# Autodesk Inventor assembly: robot_main_board
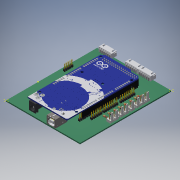
[picture p0: Inventor's stored thumbnail of the model, 180x180]
Saved by Autodesk Inventor 2019 (Build 230136000, 136)
## iProperties
Created: 2020-01-04
Part Number: robot_main_board
Material: Типовые
Document SubType Name: Assembly
Designer: Петров Иван
Author: Петров Иван
## Documents named in this file (7)
- E:\IVAN\Ivan_desktop\GitHub\Arm_manip\electronic\3d_visualization\robot_main_board\robot_main_board.iam
- E:\IVAN\Ivan_desktop\GitHub\Arm_manip\electronic\3d_visualization\robot_main_board\board.ipt
- E:\IVAN\Ivan_desktop\GitHub\Arm_manip\electronic\3d_visualization\lib\Connectors\PLS-1_(DS1021_CONNFLY).ipt
- E:\IVAN\Ivan_desktop\GitHub\Arm_manip\electronic\3d_visualization\lib\resistors\1,0 kOhm R Axial DIN0207 L6.3mm D2.5mm P7.62mm Horizontal.ipt
- E:\IVAN\Ivan_desktop\GitHub\Arm_manip\electronic\3d_visualization\lib\Connectors\JST - XH - Thru (R) - 6Pin - 2.54mm.ipt
- E:\IVAN\Ivan_desktop\GitHub\Arm_manip\electronic\3d_visualization\lib\Connectors\Molex 22-27-2021 v1.ipt
- E:\IVAN\Ivan_desktop\GitHub\Arm_manip\electronic\3d_visualization\lib\Arduino MEGA 2560 R3.ipt
## Components (151 placed, 6 different names)
1. board:1 — Совмещение:1, Совмещение:2, Угол:1, Совмещение:3, Совмещение:4, Совмещение:5, Совмещение:6, Совмещение:7, Совмещение:8, Угол:4, Угол:5, Угол:6, Совмещение:9, Совмещение:10, Угол:7, Совмещение:11, Совмещение:12, Угол:8, Совмещение:13, Угол:9, Совмещение:14, Совмещение:15, Угол:10, Совмещение:16, Совмещение:17, Угол:11, Совмещение:18, Совмещение:19, Совмещение:20, Совмещение:21, Угол:13, Совмещение:22, Совмещение:23, Угол:14, Совмещение:24, Совмещение:25, Совмещение:26, Угол:15, Совмещение:27, Угол:16, Совмещение:28, Совмещение:29, Совмещение:30, Касательность:1, Совмещение:31, Совмещение:32, Касательность:2, Совмещение:33, Совмещение:34, Касательность:3, Совмещение:35, Совмещение:36, Касательность:4, Совмещение:37, Совмещение:38, Касательность:5, Совмещение:39, Совмещение:40, Касательность:6, Совмещение:41, Совмещение:42, Касательность:7, Совмещение:43, Совмещение:44, Касательность:8, Совмещение:45, Совмещение:46, Совмещение:47, Совмещение:48, Совмещение:49, Совмещение:50, Совмещение:51, Совмещение:52, Совмещение:53, Совмещение:54, Совмещение:55, Угол:17, Совмещение:56, Угол:18, Совмещение:57, Совмещение:58, Совмещение:59, Совмещение:60, Совмещение:61, Совмещение:62, Совмещение:63, Угол:19, Угол:20, Угол:21, Угол:22, Угол:23, Угол:24, Совмещение:64, Совмещение:65, Совмещение:66, Совмещение:67, Совмещение:68, Совмещение:69
2. 1,0 kOhm R Axial DIN0207 L6.3mm D2.5mm P7.62mm Horizontal:1 — Совмещение:29, Совмещение:30, Касательность:1
3. 1,0 kOhm R Axial DIN0207 L6.3mm D2.5mm P7.62mm Horizontal:2 — Совмещение:31, Совмещение:32, Касательность:2
4. 1,0 kOhm R Axial DIN0207 L6.3mm D2.5mm P7.62mm Horizontal:3 — Совмещение:33, Совмещение:34, Касательность:3
5. 1,0 kOhm R Axial DIN0207 L6.3mm D2.5mm P7.62mm Horizontal:4 — Совмещение:35, Совмещение:36, Касательность:4
6. 1,0 kOhm R Axial DIN0207 L6.3mm D2.5mm P7.62mm Horizontal:5 — Совмещение:37, Совмещение:38, Касательность:5
7. 1,0 kOhm R Axial DIN0207 L6.3mm D2.5mm P7.62mm Horizontal:6 — Совмещение:39, Совмещение:40, Касательность:6
8. 1,0 kOhm R Axial DIN0207 L6.3mm D2.5mm P7.62mm Horizontal:7 — Совмещение:41, Совмещение:42, Касательность:7
9. 1,0 kOhm R Axial DIN0207 L6.3mm D2.5mm P7.62mm Horizontal:8 — Совмещение:43, Совмещение:44, Касательность:8
10. JST - XH - Thru (R) - 6Pin - 2.54mm:1 — Совмещение:51, Совмещение:52, Совмещение:53
11. JST - XH - Thru (R) - 6Pin - 2.54mm:2 — Совмещение:48, Совмещение:49, Совмещение:50
12. JST - XH - Thru (R) - 6Pin - 2.54mm:3 — Совмещение:45, Совмещение:46, Совмещение:47
13. Molex 22-27-2021 v1:1 — Совмещение:54, Совмещение:55, Угол:17
14. Molex 22-27-2021 v1:2 — Совмещение:56, Угол:18, Совмещение:57
15. Molex 22-27-2021 v1:3 — Совмещение:58, Угол:24, Совмещение:64
16. Molex 22-27-2021 v1:4 — Совмещение:59, Угол:23, Совмещение:65
17. Molex 22-27-2021 v1:5 — Совмещение:60, Угол:22, Совмещение:66
18. Molex 22-27-2021 v1:6 — Совмещение:61, Угол:21, Совмещение:67
19. Molex 22-27-2021 v1:7 — Совмещение:62, Угол:19, Совмещение:68
20. Molex 22-27-2021 v1:8 — Совмещение:63, Угол:20, Совмещение:69
21. Arduino MEGA 2560 R3:1 — Совмещение:70, Совмещение:72, Совмещение:73
22. PLS-1_(DS1021_CONNFLY):1 — Совмещение:1, Совмещение:2, Угол:1
23. PLS-1_(DS1021_CONNFLY):4
24. PLS-1_(DS1021_CONNFLY):5
25. PLS-1_(DS1021_CONNFLY):6
26. PLS-1_(DS1021_CONNFLY):7
27. PLS-1_(DS1021_CONNFLY):2 — Совмещение:3, Совмещение:4, Угол:5
28. PLS-1_(DS1021_CONNFLY):8
29. PLS-1_(DS1021_CONNFLY):9
30. PLS-1_(DS1021_CONNFLY):10
31. PLS-1_(DS1021_CONNFLY):11
32. PLS-1_(DS1021_CONNFLY):12
33. PLS-1_(DS1021_CONNFLY):13
34. PLS-1_(DS1021_CONNFLY):3 — Совмещение:5, Совмещение:6, Угол:6
35. PLS-1_(DS1021_CONNFLY):14
36. PLS-1_(DS1021_CONNFLY):15
37. PLS-1_(DS1021_CONNFLY):16
38. PLS-1_(DS1021_CONNFLY):17
39. PLS-1_(DS1021_CONNFLY):18 — Совмещение:7, Совмещение:8, Угол:4
40. PLS-1_(DS1021_CONNFLY):19
41. PLS-1_(DS1021_CONNFLY):20
42. PLS-1_(DS1021_CONNFLY):21
43. PLS-1_(DS1021_CONNFLY):22
44. PLS-1_(DS1021_CONNFLY):23 — Совмещение:9, Совмещение:10, Угол:7
45. PLS-1_(DS1021_CONNFLY):33
46. PLS-1_(DS1021_CONNFLY):34
47. PLS-1_(DS1021_CONNFLY):35
48. PLS-1_(DS1021_CONNFLY):36
49. PLS-1_(DS1021_CONNFLY):37
50. PLS-1_(DS1021_CONNFLY):38
51. PLS-1_(DS1021_CONNFLY):39
52. PLS-1_(DS1021_CONNFLY):24 — Совмещение:11, Совмещение:12, Угол:8
53. PLS-1_(DS1021_CONNFLY):40
54. PLS-1_(DS1021_CONNFLY):41
55. PLS-1_(DS1021_CONNFLY):42
56. PLS-1_(DS1021_CONNFLY):43
57. PLS-1_(DS1021_CONNFLY):44
58. PLS-1_(DS1021_CONNFLY):45
59. PLS-1_(DS1021_CONNFLY):46
60. PLS-1_(DS1021_CONNFLY):25 — Совмещение:13, Угол:9, Совмещение:14
61. PLS-1_(DS1021_CONNFLY):47
62. PLS-1_(DS1021_CONNFLY):48
63. PLS-1_(DS1021_CONNFLY):49
64. PLS-1_(DS1021_CONNFLY):50
65. PLS-1_(DS1021_CONNFLY):51
66. PLS-1_(DS1021_CONNFLY):52
67. PLS-1_(DS1021_CONNFLY):53
68. PLS-1_(DS1021_CONNFLY):26 — Совмещение:15, Угол:10, Совмещение:16
69. PLS-1_(DS1021_CONNFLY):54
70. PLS-1_(DS1021_CONNFLY):55
71. PLS-1_(DS1021_CONNFLY):56
72. PLS-1_(DS1021_CONNFLY):57
73. PLS-1_(DS1021_CONNFLY):58
74. PLS-1_(DS1021_CONNFLY):59
75. PLS-1_(DS1021_CONNFLY):60
76. PLS-1_(DS1021_CONNFLY):61
77. PLS-1_(DS1021_CONNFLY):62
78. PLS-1_(DS1021_CONNFLY):63
79. PLS-1_(DS1021_CONNFLY):64
80. PLS-1_(DS1021_CONNFLY):65
81. PLS-1_(DS1021_CONNFLY):66
82. PLS-1_(DS1021_CONNFLY):67
83. PLS-1_(DS1021_CONNFLY):68
84. PLS-1_(DS1021_CONNFLY):69
85. PLS-1_(DS1021_CONNFLY):70
86. PLS-1_(DS1021_CONNFLY):71
87. PLS-1_(DS1021_CONNFLY):72
88. PLS-1_(DS1021_CONNFLY):73
89. PLS-1_(DS1021_CONNFLY):74
90. PLS-1_(DS1021_CONNFLY):75
91. PLS-1_(DS1021_CONNFLY):76
92. PLS-1_(DS1021_CONNFLY):77
93. PLS-1_(DS1021_CONNFLY):78
94. PLS-1_(DS1021_CONNFLY):79
95. PLS-1_(DS1021_CONNFLY):80
96. PLS-1_(DS1021_CONNFLY):81
97. PLS-1_(DS1021_CONNFLY):82
98. PLS-1_(DS1021_CONNFLY):83
99. PLS-1_(DS1021_CONNFLY):84
100. PLS-1_(DS1021_CONNFLY):85
101. PLS-1_(DS1021_CONNFLY):86
102. PLS-1_(DS1021_CONNFLY):87
103. PLS-1_(DS1021_CONNFLY):88 — Совмещение:73
104. PLS-1_(DS1021_CONNFLY):27 — Совмещение:17, Угол:11, Совмещение:18, Угол:12, Совмещение:70
105. PLS-1_(DS1021_CONNFLY):28 — Совмещение:19, Угол:12, Совмещение:20
106. PLS-1_(DS1021_CONNFLY):30 — Совмещение:23, Угол:14, Совмещение:24
107. PLS-1_(DS1021_CONNFLY):29 — Совмещение:21, Угол:13, Совмещение:22
108. PLS-1_(DS1021_CONNFLY):89
109. PLS-1_(DS1021_CONNFLY):90
110. PLS-1_(DS1021_CONNFLY):103
111. PLS-1_(DS1021_CONNFLY):110
112. PLS-1_(DS1021_CONNFLY):91
113. PLS-1_(DS1021_CONNFLY):92
114. PLS-1_(DS1021_CONNFLY):104
115. PLS-1_(DS1021_CONNFLY):111
116. PLS-1_(DS1021_CONNFLY):93
117. PLS-1_(DS1021_CONNFLY):94
118. PLS-1_(DS1021_CONNFLY):105
119. PLS-1_(DS1021_CONNFLY):112
120. PLS-1_(DS1021_CONNFLY):95
121. PLS-1_(DS1021_CONNFLY):96
122. PLS-1_(DS1021_CONNFLY):106
123. PLS-1_(DS1021_CONNFLY):113
124. PLS-1_(DS1021_CONNFLY):97
125. PLS-1_(DS1021_CONNFLY):98
126. PLS-1_(DS1021_CONNFLY):107
127. PLS-1_(DS1021_CONNFLY):114
128. PLS-1_(DS1021_CONNFLY):99
129. PLS-1_(DS1021_CONNFLY):100
130. PLS-1_(DS1021_CONNFLY):108
131. PLS-1_(DS1021_CONNFLY):115
132. PLS-1_(DS1021_CONNFLY):101
133. PLS-1_(DS1021_CONNFLY):102
134. PLS-1_(DS1021_CONNFLY):109
135. PLS-1_(DS1021_CONNFLY):116
136. PLS-1_(DS1021_CONNFLY):31 — Совмещение:25, Совмещение:26, Угол:15
137. PLS-1_(DS1021_CONNFLY):117
138. PLS-1_(DS1021_CONNFLY):118
139. PLS-1_(DS1021_CONNFLY):119
140. PLS-1_(DS1021_CONNFLY):120
141. PLS-1_(DS1021_CONNFLY):121
142. PLS-1_(DS1021_CONNFLY):122
143. PLS-1_(DS1021_CONNFLY):123
144. PLS-1_(DS1021_CONNFLY):124
145. PLS-1_(DS1021_CONNFLY):125 — Совмещение:72
146. PLS-1_(DS1021_CONNFLY):32 — Совмещение:27, Угол:16, Совмещение:28
147. PLS-1_(DS1021_CONNFLY):126
148. PLS-1_(DS1021_CONNFLY):127
149. PLS-1_(DS1021_CONNFLY):128
150. PLS-1_(DS1021_CONNFLY):129
151. PLS-1_(DS1021_CONNFLY):130
## Component patterns: (5 elements, first: PLS-1_(DS1021_CONNFLY):1), (7 elements, first: PLS-1_(DS1021_CONNFLY):2), (5 elements, first: PLS-1_(DS1021_CONNFLY):3), (5 elements, first: PLS-1_(DS1021_CONNFLY):18), (8 elements, first: PLS-1_(DS1021_CONNFLY):23), (8 elements, first: PLS-1_(DS1021_CONNFLY):24), (8 elements, first: PLS-1_(DS1021_CONNFLY):25), (36 elements, first: PLS-1_(DS1021_CONNFLY):26), (8 elements, first: PLS-1_(DS1021_CONNFLY):27 + PLS-1_(DS1021_CONNFLY):28 + PLS-1_(DS1021_CONNFLY):30 + PLS-1_(DS1021_CONNFLY):29), (10 elements, first: PLS-1_(DS1021_CONNFLY):31), (6 elements, first: PLS-1_(DS1021_CONNFLY):32)
## Relationships (102: Mate 72, Angle 22, Tangent 8)
- Совмещение:1 [Mate]: board:1 ↔ PLS-1_(DS1021_CONNFLY):1
- Совмещение:2 [Mate]: board:1 ↔ PLS-1_(DS1021_CONNFLY):1
- Угол:1 [Angle] (90 deg): board:1 ↔ PLS-1_(DS1021_CONNFLY):1
- Совмещение:3 [Mate]: board:1 ↔ PLS-1_(DS1021_CONNFLY):2
- Совмещение:4 [Mate]: board:1 ↔ PLS-1_(DS1021_CONNFLY):2
- Совмещение:5 [Mate]: board:1 ↔ PLS-1_(DS1021_CONNFLY):3
- Совмещение:6 [Mate]: board:1 ↔ PLS-1_(DS1021_CONNFLY):3
- Совмещение:7 [Mate]: board:1 ↔ PLS-1_(DS1021_CONNFLY):18
- Совмещение:8 [Mate]: board:1 ↔ PLS-1_(DS1021_CONNFLY):18
- Угол:4 [Angle] (90 deg): board:1 ↔ PLS-1_(DS1021_CONNFLY):18
- Угол:5 [Angle] (90 deg): board:1 ↔ PLS-1_(DS1021_CONNFLY):2
- Угол:6 [Angle] (90 deg): board:1 ↔ PLS-1_(DS1021_CONNFLY):3
- Совмещение:9 [Mate]: board:1 ↔ PLS-1_(DS1021_CONNFLY):23
- Совмещение:10 [Mate]: board:1 ↔ PLS-1_(DS1021_CONNFLY):23
- Угол:7 [Angle] (0 deg): board:1 ↔ PLS-1_(DS1021_CONNFLY):23
- Совмещение:11 [Mate]: board:1 ↔ PLS-1_(DS1021_CONNFLY):24
- Совмещение:12 [Mate]: board:1 ↔ PLS-1_(DS1021_CONNFLY):24
- Угол:8 [Angle] (0 deg): board:1 ↔ PLS-1_(DS1021_CONNFLY):24
- Совмещение:13 [Mate]: board:1 ↔ PLS-1_(DS1021_CONNFLY):25
- Угол:9 [Angle] (0 deg): board:1 ↔ PLS-1_(DS1021_CONNFLY):25
- Совмещение:14 [Mate]: board:1 ↔ PLS-1_(DS1021_CONNFLY):25
- Совмещение:15 [Mate]: board:1 ↔ PLS-1_(DS1021_CONNFLY):26
- Угол:10 [Angle] (90 deg): board:1 ↔ PLS-1_(DS1021_CONNFLY):26
- Совмещение:16 [Mate]: board:1 ↔ PLS-1_(DS1021_CONNFLY):26
- Совмещение:17 [Mate]: board:1 ↔ PLS-1_(DS1021_CONNFLY):27
- Угол:11 [Angle] (0 deg): board:1 ↔ PLS-1_(DS1021_CONNFLY):27
- Совмещение:18 [Mate]: board:1 ↔ PLS-1_(DS1021_CONNFLY):27
- Совмещение:19 [Mate]: board:1 ↔ PLS-1_(DS1021_CONNFLY):28
- Угол:12 [Angle] (90 deg): PLS-1_(DS1021_CONNFLY):27 ↔ PLS-1_(DS1021_CONNFLY):28
- Совмещение:20 [Mate]: board:1 ↔ PLS-1_(DS1021_CONNFLY):28
- Совмещение:21 [Mate]: board:1 ↔ PLS-1_(DS1021_CONNFLY):29
- Угол:13 [Angle] (90 deg): board:1 ↔ PLS-1_(DS1021_CONNFLY):29
- Совмещение:22 [Mate]: board:1 ↔ PLS-1_(DS1021_CONNFLY):29
- Совмещение:23 [Mate]: board:1 ↔ PLS-1_(DS1021_CONNFLY):30
- Угол:14 [Angle] (0 deg): board:1 ↔ PLS-1_(DS1021_CONNFLY):30
- Совмещение:24 [Mate]: board:1 ↔ PLS-1_(DS1021_CONNFLY):30
- Совмещение:25 [Mate]: board:1 ↔ PLS-1_(DS1021_CONNFLY):31
- Совмещение:26 [Mate]: board:1 ↔ PLS-1_(DS1021_CONNFLY):31
- Угол:15 [Angle] (0 deg): board:1 ↔ PLS-1_(DS1021_CONNFLY):31
- Совмещение:27 [Mate]: board:1 ↔ PLS-1_(DS1021_CONNFLY):32
- Угол:16 [Angle] (90 deg): board:1 ↔ PLS-1_(DS1021_CONNFLY):32
- Совмещение:28 [Mate]: board:1 ↔ PLS-1_(DS1021_CONNFLY):32
- Совмещение:29 [Mate]: board:1 ↔ 1,0 kOhm R Axial DIN0207 L6.3mm D2.5mm P7.62mm Horizontal:1
- Совмещение:30 [Mate]: board:1 ↔ 1,0 kOhm R Axial DIN0207 L6.3mm D2.5mm P7.62mm Horizontal:1
- Касательность:1 [Tangent]: board:1 ↔ 1,0 kOhm R Axial DIN0207 L6.3mm D2.5mm P7.62mm Horizontal:1
- Совмещение:31 [Mate]: board:1 ↔ 1,0 kOhm R Axial DIN0207 L6.3mm D2.5mm P7.62mm Horizontal:2
- Совмещение:32 [Mate]: board:1 ↔ 1,0 kOhm R Axial DIN0207 L6.3mm D2.5mm P7.62mm Horizontal:2
- Касательность:2 [Tangent]: board:1 ↔ 1,0 kOhm R Axial DIN0207 L6.3mm D2.5mm P7.62mm Horizontal:2
- Совмещение:33 [Mate]: board:1 ↔ 1,0 kOhm R Axial DIN0207 L6.3mm D2.5mm P7.62mm Horizontal:3
- Совмещение:34 [Mate]: board:1 ↔ 1,0 kOhm R Axial DIN0207 L6.3mm D2.5mm P7.62mm Horizontal:3
- Касательность:3 [Tangent]: board:1 ↔ 1,0 kOhm R Axial DIN0207 L6.3mm D2.5mm P7.62mm Horizontal:3
- Совмещение:35 [Mate]: board:1 ↔ 1,0 kOhm R Axial DIN0207 L6.3mm D2.5mm P7.62mm Horizontal:4
- Совмещение:36 [Mate]: board:1 ↔ 1,0 kOhm R Axial DIN0207 L6.3mm D2.5mm P7.62mm Horizontal:4
- Касательность:4 [Tangent]: board:1 ↔ 1,0 kOhm R Axial DIN0207 L6.3mm D2.5mm P7.62mm Horizontal:4
- Совмещение:37 [Mate]: board:1 ↔ 1,0 kOhm R Axial DIN0207 L6.3mm D2.5mm P7.62mm Horizontal:5
- Совмещение:38 [Mate]: board:1 ↔ 1,0 kOhm R Axial DIN0207 L6.3mm D2.5mm P7.62mm Horizontal:5
- Касательность:5 [Tangent]: board:1 ↔ 1,0 kOhm R Axial DIN0207 L6.3mm D2.5mm P7.62mm Horizontal:5
- Совмещение:39 [Mate]: board:1 ↔ 1,0 kOhm R Axial DIN0207 L6.3mm D2.5mm P7.62mm Horizontal:6
- Совмещение:40 [Mate]: board:1 ↔ 1,0 kOhm R Axial DIN0207 L6.3mm D2.5mm P7.62mm Horizontal:6
- Касательность:6 [Tangent]: board:1 ↔ 1,0 kOhm R Axial DIN0207 L6.3mm D2.5mm P7.62mm Horizontal:6
- Совмещение:41 [Mate]: board:1 ↔ 1,0 kOhm R Axial DIN0207 L6.3mm D2.5mm P7.62mm Horizontal:7
- Совмещение:42 [Mate]: board:1 ↔ 1,0 kOhm R Axial DIN0207 L6.3mm D2.5mm P7.62mm Horizontal:7
- Касательность:7 [Tangent]: board:1 ↔ 1,0 kOhm R Axial DIN0207 L6.3mm D2.5mm P7.62mm Horizontal:7
- Совмещение:43 [Mate]: board:1 ↔ 1,0 kOhm R Axial DIN0207 L6.3mm D2.5mm P7.62mm Horizontal:8
- Совмещение:44 [Mate]: board:1 ↔ 1,0 kOhm R Axial DIN0207 L6.3mm D2.5mm P7.62mm Horizontal:8
- Касательность:8 [Tangent]: board:1 ↔ 1,0 kOhm R Axial DIN0207 L6.3mm D2.5mm P7.62mm Horizontal:8
- Совмещение:45 [Mate]: board:1 ↔ JST - XH - Thru (R) - 6Pin - 2.54mm:3
- Совмещение:46 [Mate]: board:1 ↔ JST - XH - Thru (R) - 6Pin - 2.54mm:3
- Совмещение:47 [Mate]: board:1 ↔ JST - XH - Thru (R) - 6Pin - 2.54mm:3
- Совмещение:48 [Mate]: board:1 ↔ JST - XH - Thru (R) - 6Pin - 2.54mm:2
- Совмещение:49 [Mate]: board:1 ↔ JST - XH - Thru (R) - 6Pin - 2.54mm:2
- Совмещение:50 [Mate]: board:1 ↔ JST - XH - Thru (R) - 6Pin - 2.54mm:2
- Совмещение:51 [Mate]: board:1 ↔ JST - XH - Thru (R) - 6Pin - 2.54mm:1
- Совмещение:52 [Mate]: board:1 ↔ JST - XH - Thru (R) - 6Pin - 2.54mm:1
- Совмещение:53 [Mate]: board:1 ↔ JST - XH - Thru (R) - 6Pin - 2.54mm:1
- Совмещение:54 [Mate]: board:1 ↔ Molex 22-27-2021 v1:1
- Совмещение:55 [Mate]: board:1 ↔ Molex 22-27-2021 v1:1
- Угол:17 [Angle] (0 deg): board:1 ↔ Molex 22-27-2021 v1:1
- Совмещение:56 [Mate]: board:1 ↔ Molex 22-27-2021 v1:2
- Угол:18 [Angle] (0 deg): board:1 ↔ Molex 22-27-2021 v1:2
- Совмещение:57 [Mate]: board:1 ↔ Molex 22-27-2021 v1:2
- Совмещение:58 [Mate]: board:1 ↔ Molex 22-27-2021 v1:3
- Совмещение:59 [Mate]: board:1 ↔ Molex 22-27-2021 v1:4
- Совмещение:60 [Mate]: board:1 ↔ Molex 22-27-2021 v1:5
- Совмещение:61 [Mate]: board:1 ↔ Molex 22-27-2021 v1:6
- Совмещение:62 [Mate]: board:1 ↔ Molex 22-27-2021 v1:7
- Совмещение:63 [Mate]: board:1 ↔ Molex 22-27-2021 v1:8
- Угол:19 [Angle] (0 deg): board:1 ↔ Molex 22-27-2021 v1:7
- Угол:20 [Angle] (0 deg): board:1 ↔ Molex 22-27-2021 v1:8
- Угол:21 [Angle] (0 deg): board:1 ↔ Molex 22-27-2021 v1:6
- Угол:22 [Angle] (0 deg): board:1 ↔ Molex 22-27-2021 v1:5
- Угол:23 [Angle] (0 deg): board:1 ↔ Molex 22-27-2021 v1:4
- Угол:24 [Angle] (0 deg): board:1 ↔ Molex 22-27-2021 v1:3
- Совмещение:64 [Mate]: board:1 ↔ Molex 22-27-2021 v1:3
- Совмещение:65 [Mate]: board:1 ↔ Molex 22-27-2021 v1:4
- Совмещение:66 [Mate]: board:1 ↔ Molex 22-27-2021 v1:5
- Совмещение:67 [Mate]: board:1 ↔ Molex 22-27-2021 v1:6
- Совмещение:68 [Mate]: board:1 ↔ Molex 22-27-2021 v1:7
- Совмещение:69 [Mate]: board:1 ↔ Molex 22-27-2021 v1:8
- Совмещение:70 [Mate]: Arduino MEGA 2560 R3:1 ↔ PLS-1_(DS1021_CONNFLY):27
- Совмещение:72 [Mate]: Arduino MEGA 2560 R3:1 ↔ PLS-1_(DS1021_CONNFLY):125
- Совмещение:73 [Mate]: Arduino MEGA 2560 R3:1 ↔ PLS-1_(DS1021_CONNFLY):88
